# Autodesk Inventor assembly: inner
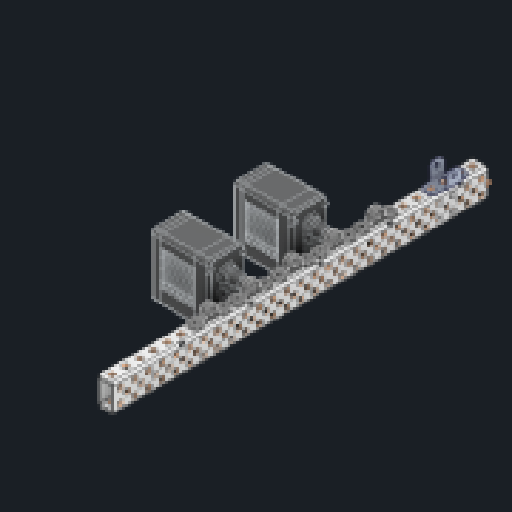
[picture p0: Inventor's stored thumbnail of the model, 512x512]
Saved by Autodesk Inventor 2024 (Build 280153000, 153)
## iProperties
Created: 2023-08-15
Part Number: inner
Document SubType Name: Assembly
Designer: avere
Author: avere
## Documents named in this file (14)
- D:\cad\scrap_v0.1\chassis\inner.iam
- D:\cad\VEX-CAD-Inventor-1.41\Structure\C Channel\Aluminum 1x2x1\Alu C 1x2x1x27.ipt
- D:\cad\VEX-CAD-Inventor-1.41\Motion\Shaft LS\LS Pillow Bearing Block.ipt
- D:\cad\VEX-CAD-Inventor-1.41\Electronics\V5 Motor.ipt
- D:\cad\VEX-CAD-Inventor-1.41\Motion\Spacers\Spacer Nylon .375 OD\NSpacer .375 OD x .125.ipt
- D:\cad\VEX-CAD-Inventor-1.41\Motion\Spacers\Spacer Nylon .375 OD\NSpacer .375 OD x .500.ipt
- D:\cad\VEX-CAD-Inventor-1.41\Structure\4-Post Hex Nut Retainer.ipt
- D:\cad\VEX-CAD-Inventor-1.41\Motion\Shaft LS\Bearing Flat.ipt
- D:\cad\VEX-CAD-Inventor-1.41\Structure\Gussets\C Channel Coupler.ipt
- D:\cad\VEX-CAD-Inventor-1.41\Motion\Gears\LS 12T Gear Steel.ipt
- D:\cad\VEX-CAD-Inventor-1.41\Motion\Shaft LS\Bearing Flat Low Profile.ipt
- D:\cad\VEX-CAD-Inventor-1.41\Motion\Spacers\Spacer Nylon .375 OD\NSpacer .375 OD x .250.ipt
- D:\cad\VEX-CAD-Inventor-1.41\Motion\Spacers\Spacer Nylon .375 OD.ipt
- D:\cad\VEX-CAD-Inventor-1.41\Motion\Pneumatics\Cylinder Rod Pivot.ipt
## Components (22 placed, 12 different names)
1. Alu C 1x2x1x27:1 — Insert:30, Mate:15, Insert:35, Mate:16, Insert:36, Mate:17, Insert:45, Insert:54, Mate:24, Insert:55, Mate:25, Insert:57, Mate:27, Insert:58, Mate:28, Insert:61, Mate:29, Insert:65, Mate:30, Insert:66, Insert:67, Mate:31, Insert:68, Mate:32
2. LS Pillow Bearing Block:4 — Insert:54, Mate:24
3. 4-Post Hex Nut Retainer:2 — Insert:30, Mate:15
4. Bearing Flat:1 — Insert:35, Mate:16
5. C Channel Coupler:1 — Insert:36, Mate:17
6. LS Pillow Bearing Block:7 — Insert:64, Insert:65, Mate:30
7. LS 12T Gear Steel:1 — Insert:63
8. V5 Motor:10 — Insert:47, Insert:48
9. NSpacer .375 OD x .500:16 — Insert:48, Insert:66
10. NSpacer .375 OD x .125:17 — Insert:47, Insert:64
11. LS Pillow Bearing Block:9 — Insert:45
12. V5 Motor:11
13. NSpacer .375 OD x .500:18
14. NSpacer .375 OD x .125:19
15. LS Pillow Bearing Block:10 — Insert:55, Mate:25
16. Bearing Flat Low Profile:1 — Insert:57, Mate:27
17. Bearing Flat Low Profile:2 — Insert:58, Mate:28, Insert:60
18. Bearing Flat Low Profile:3 — Insert:61, Mate:29
19. NSpacer .375 OD x .250:20 — Insert:60, Insert:62
20. NSpacer .375 OD x .250:21 — Insert:62, Insert:63
21. LS Pillow Bearing Block:11 — Insert:67, Mate:31
22. Cylinder Rod Pivot:1 — Insert:68, Mate:32
## Relationships (33: Insert 22, Mate 11)
- Insert:30: Alu C 1x2x1x27:1 ↔ 4-Post Hex Nut Retainer:2
- Mate:15: Alu C 1x2x1x27:1 ↔ 4-Post Hex Nut Retainer:2
- Insert:35: Alu C 1x2x1x27:1 ↔ Bearing Flat:1
- Mate:16: Alu C 1x2x1x27:1 ↔ Bearing Flat:1
- Insert:36: Alu C 1x2x1x27:1 ↔ C Channel Coupler:1
- Mate:17: Alu C 1x2x1x27:1 ↔ C Channel Coupler:1
- Insert:45: Alu C 1x2x1x27:1 ↔ LS Pillow Bearing Block:9
- Insert:47: V5 Motor:10 ↔ NSpacer .375 OD x .125:17
- Insert:48: V5 Motor:10 ↔ NSpacer .375 OD x .500:16
- [Insert]: NSpacer .375 OD x .125:19 ↔ LS Pillow Bearing Block:10
- [Insert]: V5 Motor:11 ↔ NSpacer .375 OD x .125:19
- [Insert]: V5 Motor:11 ↔ NSpacer .375 OD x .500:18
- Insert:54: Alu C 1x2x1x27:1 ↔ LS Pillow Bearing Block:4
- Mate:24: Alu C 1x2x1x27:1 ↔ LS Pillow Bearing Block:4
- Insert:55: Alu C 1x2x1x27:1 ↔ LS Pillow Bearing Block:10
- Mate:25: Alu C 1x2x1x27:1 ↔ LS Pillow Bearing Block:10
- Insert:57: Alu C 1x2x1x27:1 ↔ Bearing Flat Low Profile:1
- Mate:27: Alu C 1x2x1x27:1 ↔ Bearing Flat Low Profile:1
- Insert:58: Alu C 1x2x1x27:1 ↔ Bearing Flat Low Profile:2
- Mate:28: Alu C 1x2x1x27:1 ↔ Bearing Flat Low Profile:2
- Insert:60 (1.27 mm): Bearing Flat Low Profile:2 ↔ NSpacer .375 OD x .250:20
- Insert:61: Alu C 1x2x1x27:1 ↔ Bearing Flat Low Profile:3
- Mate:29: Alu C 1x2x1x27:1 ↔ Bearing Flat Low Profile:3
- Insert:62: NSpacer .375 OD x .250:20 ↔ NSpacer .375 OD x .250:21
- Insert:63: LS 12T Gear Steel:1 ↔ NSpacer .375 OD x .250:21
- Insert:64: LS Pillow Bearing Block:7 ↔ NSpacer .375 OD x .125:17
- Insert:65: Alu C 1x2x1x27:1 ↔ LS Pillow Bearing Block:7
- Mate:30: Alu C 1x2x1x27:1 ↔ LS Pillow Bearing Block:7
- Insert:66: Alu C 1x2x1x27:1 ↔ NSpacer .375 OD x .500:16
- Insert:67: Alu C 1x2x1x27:1 ↔ LS Pillow Bearing Block:11
- Mate:31: Alu C 1x2x1x27:1 ↔ LS Pillow Bearing Block:11
- Insert:68: Alu C 1x2x1x27:1 ↔ Cylinder Rod Pivot:1
- Mate:32: Alu C 1x2x1x27:1 ↔ Cylinder Rod Pivot:1
## Named parameters: d74_d70 = 0 mm, d75_d71 = 0 mm, d76_d72 = 0 mm
